# Autodesk Inventor assembly: Assembly
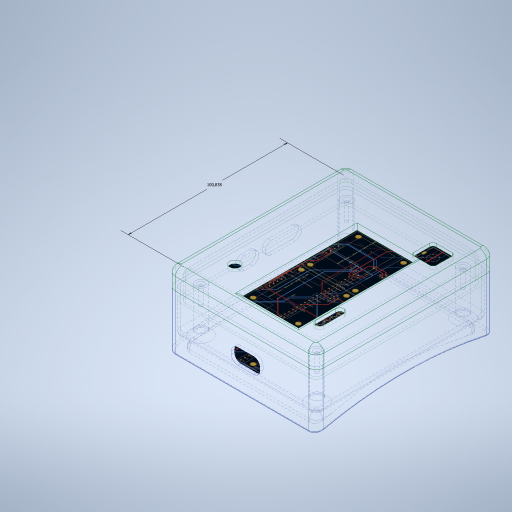
[picture p0: Inventor's stored thumbnail of the model, 512x512]
Saved by Autodesk Inventor 2024.4 (Build 284460000, 460)
## iProperties
Created: 2026-05-24
Part Number: Assembly
Document SubType Name: Assembly
Designer: Emil
Author: Emil
## Documents named in this file (4)
- C:\Users\Emil\OneDrive\Dokument\Projekt-Emil\MachMachine\InventorCad\Lautering Tank box V2.0\Assembly.iam
- C:\Users\Emil\OneDrive\Dokument\Projekt-Emil\MachMachine\InventorCad\Lautering Tank box V2.0\lautering_tank_box.ipt
- lautering_tank_box_base.ipt
- C:\Users\Emil\OneDrive\Dokument\Projekt-Emil\MachMachine\InventorCad\Lautering Tank box V2.0\lid_lautering_tank.ipt
## Components (2 placed, 2 different names)
1. lautering_tank_box_base:1 — Mate:1, Flush:1, Flush:2
2. lid_lautering_tank:1 — Mate:1, Flush:1, Flush:2
## Relationships (3: Flush 2, Mate 1)
- Mate:1: lautering_tank_box_base:1 ↔ lid_lautering_tank:1
- Flush:1: lautering_tank_box_base:1 ↔ lid_lautering_tank:1
- Flush:2: lautering_tank_box_base:1 ↔ lid_lautering_tank:1
